# Autodesk Inventor assembly: screw_MIR
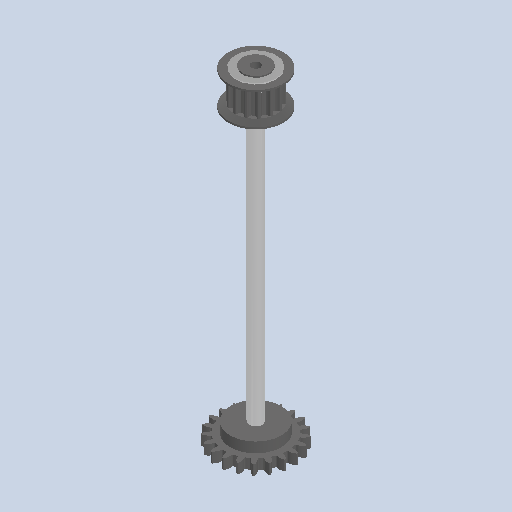
[picture p0: Inventor's stored thumbnail of the model, 512x512]
Saved by Autodesk Inventor 2024.1 (Build 281209000, 209)
## iProperties
Created: 2025-01-17
Part Number: screw_MIR
Document SubType Name: Assembly
Designer: hibik
Author: hibik
## Documents named in this file (6)
- C:\Users\hibik\Documents\Robomech\RESCUE\ORCA\hard\fork\right\screw_MIR.iam
- C:\Users\hibik\Documents\Robomech\RESCUE\ORCA\hard\fork\right\screw_screw_MIR.ipt
- C:\Users\hibik\Documents\Robomech\RESCUE\ORCA\hard\fork\right\screw_gear_upper_MIR.ipt
- C:\Users\hibik\Documents\Robomech\RESCUE\ORCA\hard\fork\right\screw_gear_under_MIR.ipt
- C:\Users\hibik\Documents\Robomech\RESCUE\ORCA\hard\std_parts\bearing_6_10_3_MIR.ipt
- C:\Users\hibik\Documents\Robomech\RESCUE\ORCA\hard\fork\right\screw_bearing_setter_MIR.ipt
## Components (7 placed, 5 different names)
1. screw_screw_MIR:1 — 挿入:2, 挿入:3
2. screw_gear_upper_MIR:1 — 挿入:2, 挿入:4
3. screw_gear_under_MIR:1 — 挿入:3, 挿入:5
4. bearing_6_10_3_MIR:1 — 挿入:4, 挿入:7
5. bearing_6_10_3_MIR:2 — 挿入:5, 挿入:6
6. screw_bearing_setter_MIR:1 — 挿入:6
7. screw_bearing_setter_MIR:2 — 挿入:7
## Relationships (6: Insert 6)
- 挿入:2 [Insert]: screw_screw_MIR:1 ↔ screw_gear_upper_MIR:1
- 挿入:3 [Insert]: screw_screw_MIR:1 ↔ screw_gear_under_MIR:1
- 挿入:4 [Insert]: screw_gear_upper_MIR:1 ↔ bearing_6_10_3_MIR:1
- 挿入:5 [Insert]: screw_gear_under_MIR:1 ↔ bearing_6_10_3_MIR:2
- 挿入:6 [Insert]: bearing_6_10_3_MIR:2 ↔ screw_bearing_setter_MIR:1
- 挿入:7 [Insert]: bearing_6_10_3_MIR:1 ↔ screw_bearing_setter_MIR:2
